# Autodesk Inventor assembly: Ensamblaje3
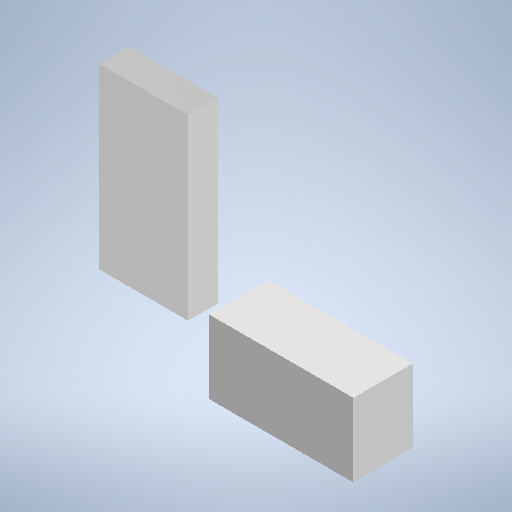
[picture p0: Inventor's stored thumbnail of the model, 512x512]
Saved by Autodesk Inventor 2025.2 (Build 292293000, 293)
## iProperties
Created: 2025-01-20
Part Number: Ensamblaje3
Document SubType Name: Assembly
Designer: usuario
Author: usuario
## Documents named in this file (3)
- C:\Users\usuario\Desktop\ModeladosAPM\MOTO\Ensamblaje3.iam
- C:\Users\usuario\Desktop\ModeladosAPM\MOTO\Ensamblaje1.ipt
- C:\Users\usuario\Desktop\ModeladosAPM\MOLDES BARCO\MoldeIzquierdoPiezaInferiorBarco.ipt
## Components (2 placed, 2 different names)
1. Ensamblaje1:1 — Coincidencia:1
2. MoldeIzquierdoPiezaInferiorBarco:1 — Coincidencia:1
## Relationships (1: Mate 1)
- Coincidencia:1 [Mate]: Ensamblaje1:1 ↔ MoldeIzquierdoPiezaInferiorBarco:1
